# Autodesk Inventor assembly: FinalAssembly
(part 2 of 3)
590. ORingA70_.176ID_.316OD:12
## Component patterns: (4 elements, first: Bolt_ButtonHead_Hex_Thread_5_40_1inch:1), (6 elements, first: NarrowHexNutThread_5_40:5), (4 elements, first: NarrowHexNutThread_5_40:3), (6 elements, first: NarrowHexNutThread_5_40:14), (4 elements, first: ORingA50_.25OD_.125ID:24), (4 elements, first: Bolt_Buttonhead_Hex_Thread_5_40_.625inch:1), (4 elements, first: NarrowHexNutThread_5_40:20), (6 elements, first: ScrewPlastic_4_20_.75inch_Flat:1), (6 elements, first: NarrowHexNutThread_5_40:24), (2 elements), (2 elements), (2 elements), (6 elements, first: ORingA50_.25OD_.125ID:34), (6 elements, first: NarrowHexNutThread_5_40:50), (6 elements, first: aftThreadedRodThread_5_40:1), (6 elements, first: NarrowHexNutThread_5_40:56), (6 elements, first: ScrewPlastic_4_20_.75inch_Flat:19), (6 elements, first: NarrowHexNutThread_5_40:66), (3 elements, first: ScrewPlastic_4_20_.5inch:18), (6 elements, first: ORingA50_.25OD_.125ID:40), (6 elements, first: Bolt_Buttonhead_Hex_Thread_5_40_.625inch:5), (6 elements, first: NarrowHexNutThread_5_40:72), (6 elements, first: ORingA50_.25OD_.125ID:46), (2 elements), (6 elements, first: NarrowHexNutThread_5_40:84), (6 elements, first: midshipsThreadedRodThread_5_40:1), (6 elements, first: NarrowHexNutThread_5_40:90), (4 elements, first: flatPlasticScrewSmall:21), (6 elements, first: retentionStandoffs:1), (6 elements, first: NarrowHexNutThread_5_40:99), (3 elements, first: flatPlasticScrewSmall:36), (6 elements, first: ORingA50_.25OD_.125ID:52), (6 elements, first: NarrowHexNutThread_5_40:105), (6 elements, first: NarrowHexNutThread_5_40:111), (4 elements, first: ScrewPlastic_4_20_.5inch:25), (6 elements, first: NarrowHexNutThread_5_40:117), (6 elements, first: Bolt_Buttonhead_Hex_Thread_5_40_.625inch:11), (6 elements, first: flatPlasticScrewSmall:54), (3 elements, first: NarrowHexNutThread_5_40:135), (3 elements, first: NarrowHexNutThread_5_40:159), (3 elements, first: NarrowHexNutThread_5_40:165), (6 elements, first: aftServoSectionThreadedRodThread_5_40:1 + NarrowHexNutThread_5_40:175 + ORingA50_.25OD_.125ID:72 + NarrowHexNutThread_5_40:176), (6 elements, first: NarrowHexNutCaps:1), (4 elements, first: ScrewPlastic_4_20_.5inch:34), (3 elements, first: HexNutThread_M3:1), (6 elements, first: ORingA50_.25OD_.125ID:79 + Bolt_ButtonHead_Hex_Thread_5_40_1inch:5 + ORingA50_.25OD_.125ID:80), (3 elements, first: Bolt_ButtonHead_Hex_Thread_M3_10mm:1), (4 elements, first: EncoderMagnet:3), (2 elements, first: RelayModule:1), (3 elements, first: batteryHolderBracket:2), (3 elements, first: NarrowHexNutThread_5_40:216 + NarrowHexNutThread_5_40:215 + NarrowHexNutThread_5_40:218 + NarrowHexNutThread_5_40:217), (6 elements, first: NarrowHexNutThread_5_40:227), (3 elements, first: NarrowHexNutThread_5_40:233), (2 elements, first: NarrowHexNutThread_5_40:236 + NarrowHexNutThread_5_40:239 + NarrowHexNutThread_5_40:237 + NarrowHexNutThread_5_40:238), (4 elements, first: ScrewPlastic_4_20_.5inch:2), Component Pattern 27:2 (4 elements), (3 elements, first: ORingA70_.176ID_.316OD:1), Component Pattern 30:2 (3 elements), (3 elements, first: aluminumWiringTubing:1), Component Pattern 32:2 (3 elements), (3 elements, first: ORingA70_.176ID_.316OD:7), Component Pattern 50:2 (3 elements)
## Relationships (810: Mate 614, Flush 81, Angle 73, WeldJoint 21, RelateRotation 10, Tangent 6, BallJoint 4, RelateRotateTranslate 1)
- Mate:1: AftSectionAirtightRear:1 ↔ AftSectionWithSteeringLinkages:1
- Mate:5: AftSectionAirtightRear:1 ↔ aftSectionAirtightCap:2
- Mate:6: AftSectionAirtightRear:1 ↔ aftSectionAirtightCap:2
- Mate:8: AluminumSealingDisc:1 ↔ aftSectionAirtightCap:2
- Mate:10: AluminumSealingDisc:1 ↔ aftSectionAirtightCap:2
- Mate:11: AluminumSealingDisc:1 ↔ rearServoAttachmentPlate:1
- Mate:12: AluminumSealingDisc:1 ↔ rearServoAttachmentPlate:1
- Mate:13: AluminumSealingDisc:1 ↔ rearServoAttachmentPlate:1
- Mate:14: rearServoAttachmentPlate:1 ↔ HitecServoAssembly:1
- Mate:16: rearServoAttachmentPlate:1 ↔ HitecServoAssembly:1
- Mate:17: rearServoAttachmentPlate:1 ↔ HitecServoAssembly:2
- Mate:18: rearServoAttachmentPlate:1 ↔ HitecServoAssembly:2
- Mate:19: rearServoAttachmentPlate:1 ↔ HitecServoAssembly:2
- Mate:20: HitecServoAssembly:1 ↔ ServoHorn10mmPitch:1
- Mate:21: HitecServoAssembly:2 ↔ ServoHorn10mmPitch:2
- Mate:22: HitecServoAssembly:2 ↔ ServoHorn10mmPitch:2
- Mate:23: HitecServoAssembly:1 ↔ ServoHorn10mmPitch:1
- [Mate]: RearmostAftSection:2 ↔ steeringYoke3mmShaft:4
- [Mate]: RearmostAftSection:2 ↔ steeringYoke3mmShaft:3
- Mate:28 (7.747 mm): RearmostAftSection:2 ↔ steeringYoke3mmShaft:4
- Mate:29 (2.8575 mm): RearmostAftSection:2 ↔ steeringYoke3mmShaft:3
- Mate:30: AftSectionWithSteeringLinkages:1 ↔ RearmostAftSection:2
- Mate:31: AftSectionWithSteeringLinkages:1 ↔ RearmostAftSection:2
- Mate:36: ServoHorn10mmPitch:2 ↔ metalClevisis:5
- Mate:37: ServoHorn10mmPitch:1 ↔ metalClevisis:6
- Mate:55: metalClevisis:6 ↔ 2mmToServo:7
- Mate:56: metalClevisis:6 ↔ 2mmToServo:7
- Mate:59: steeringYoke3mmShaft:3 ↔ metalClevisis:7
- Mate:60 (0.762 mm): steeringYoke3mmShaft:3 ↔ metalClevisis:7
- Mate:61: steeringYoke3mmShaft:4 ↔ metalClevisis:8
- Ball:1: 2mmToDive:1 ↔ 2mmBentFromSealDive:2
- Mate:69: metalClevisis:7 ↔ 2mmBentFromSealDive:2
- Mate:70: metalClevisis:7 ↔ 2mmBentFromSealDive:2
- Ball:2: 2mmToSeal:4 ↔ 2mmToServo:8
- Mate:71: metalClevisis:5 ↔ 2mmToServo:8
- Mate:72: metalClevisis:5 ↔ 2mmToServo:8
- Ball:3: 2mmToServo:7 ↔ 2mmToSeal:5
- Ball:4: 2mmToRudder:1 ↔ 2mmBentFromSealRudder:2
- Mate:75: metalClevisis:8 ↔ 2mmBentFromSealRudder:2
- Mate:76: metalClevisis:8 ↔ 2mmBentFromSealRudder:2
- Mate:77 (0.762 mm): steeringYoke3mmShaft:4 ↔ metalClevisis:8
- Mate:101: AftSectionAirtightRear:1 ↔ aftSectionAirtightCap:2
- Mate:102: AluminumSealingDisc:1 ↔ aftSectionAirtightCap:2
- Angle:4 (10 deg): HitecServoAssembly:2 ↔ ServoHorn10mmPitch:2
- Angle:5 (-11 deg): HitecServoAssembly:1 ↔ ServoHorn10mmPitch:1
- Flush:6 (-1.016 mm): metalClevisis:8 ↔ YokeDowelPins:1
- Flush:7 (-1.016 mm): metalClevisis:7 ↔ YokeDowelPins:2
- Mate:109: RearmostAftSection:2 ↔ RudderStabilizingLowerFins:1
- Mate:110 (0.4445 mm): RearmostAftSection:2 ↔ RudderStabilizingLowerFins:1
- Mate:111: RearmostAftSection:2 ↔ RudderStabilizingLowerFins:1
- Mate:112: RearmostAftSection:2 ↔ RudderStabilizingLowerFins:2
- Mate:113: RearmostAftSection:2 ↔ RudderStabilizingLowerFins:2
- Mate:114 (0.4445 mm): RearmostAftSection:2 ↔ RudderStabilizingLowerFins:2
- Mate:118: RearmostAftSection:2 ↔ RudderStabilizingLowerFins:4
- Mate:119: RearmostAftSection:2 ↔ RudderStabilizingLowerFins:4
- Mate:120 (0.4445 mm): RearmostAftSection:2 ↔ RudderStabilizingLowerFins:4
- Mate:121: RearmostAftSection:2 ↔ SleeveBearing3mmFlanged:1
- Mate:122: RearmostAftSection:2 ↔ SleeveBearing3mmFlanged:1
- Mate:123: RearmostAftSection:2 ↔ SleeveBearing3mmFlanged:4
- Mate:124: RearmostAftSection:2 ↔ SleeveBearing3mmFlanged:4
- Mate:125: RearmostAftSection:2 ↔ SleeveBearing3mmFlanged:3
- Mate:126: RearmostAftSection:2 ↔ SleeveBearing3mmFlanged:3
- Mate:127: RearmostAftSection:2 ↔ SleeveBearing3mmFlanged:2
- Mate:128: RearmostAftSection:2 ↔ SleeveBearing3mmFlanged:2
- Mate:129: RearmostAftSection:2 ↔ DivePlanesStabilizingFins:1
- Mate:130: RearmostAftSection:2 ↔ DivePlanesStabilizingFins:2
- Mate:131: RearmostAftSection:2 ↔ DivePlanesStabilizingFins:2
- Mate:132: RearmostAftSection:2 ↔ DivePlanesStabilizingFins:2
- Mate:133: RearmostAftSection:2 ↔ DivePlanesStabilizingFins:1
- Mate:134: RearmostAftSection:2 ↔ DivePlanesStabilizingFins:1
- Mate:135: RearmostAftSection:2 ↔ RudderStabilizingFins:1
- Mate:136: RearmostAftSection:2 ↔ RudderStabilizingFins:1
- Angle:6 (0 deg): RearmostAftSection:2 ↔ RudderStabilizingFins:1
- Mate:137: RearmostAftSection:2 ↔ RudderStabilizingFinBottom:1
- Mate:138: RearmostAftSection:2 ↔ RudderStabilizingFinBottom:1
- Angle:7 (0 deg): RearmostAftSection:2 ↔ RudderStabilizingFinBottom:1
- Mate:139: SleeveBearing3mmFlanged:2 ↔ 3mmControlSurfaceShaft_1:1
- Mate:140: SleeveBearing3mmFlanged:4 ↔ 3mmControlSurfaceShaft_1:2
- Mate:141: SleeveBearing3mmFlanged:1 ↔ 3mmControlSurfaceShaft_2:1
- Mate:142: SleeveBearing3mmFlanged:3 ↔ 3mmControlSurfaceShaft_2:2
- Mate:143: 3mmControlSurfaceShaft_1:1 ↔ DivePlanesControlSurface:1
- Mate:144: 3mmControlSurfaceShaft_1:1 ↔ DivePlanesControlSurface:1
- Mate:147: 3mmControlSurfaceShaft_1:2 ↔ DivePlanesControlSurface:2
- Mate:148 (0.635 mm): DivePlanesStabilizingFins:2 ↔ DivePlanesControlSurface:2
- Mate:149: DivePlanesControlSurface:1 ↔ DivePlanesControlSurface:2
- Mate:150: 3mmControlSurfaceShaft_1:2 ↔ DivePlanesControlSurface:2
- Flush:8 (-0.762 mm): steeringYoke3mmShaft:3 ↔ 3mmControlSurfaceShaft_1:2
- Flush:9 (-0.762 mm): steeringYoke3mmShaft:3 ↔ 3mmControlSurfaceShaft_1:1
- Rigid:1 [WeldJoint] (-0.762 mm): steeringYoke3mmShaft:3 ↔ 3mmControlSurfaceShaft_1:1
- Mate:153: 3mmControlSurfaceShaft_2:1 ↔ RudderUpperControlSurface:1
- Mate:154: 3mmControlSurfaceShaft_2:1 ↔ RudderUpperControlSurface:1
- Mate:155: 3mmControlSurfaceShaft_2:2 ↔ RudderLowerControlSurface:1
- Mate:156: 3mmControlSurfaceShaft_2:2 ↔ RudderLowerControlSurface:1
- Mate:158 (0.254 mm): RudderStabilizingLowerFins:2 ↔ RudderLowerControlSurface:1
- Mate:159: RudderLowerControlSurface:1 ↔ RudderUpperControlSurface:1
- Rigid:2 [WeldJoint] (-1.016 mm): steeringYoke3mmShaft:4 ↔ 3mmControlSurfaceShaft_2:1
- Mate:160: RearmostAftSection:2 ↔ ScrewPlastic_4_20_.625inch:1
- Mate:161: RearmostAftSection:2 ↔ ScrewPlastic_4_20_.625inch:1
- Mate:162: RearmostAftSection:2 ↔ ScrewPlastic_4_20_.625inch:2
- Mate:163: RearmostAftSection:2 ↔ ScrewPlastic_4_20_.625inch:2
- Mate:164: RearmostAftSection:2 ↔ ScrewPlastic_4_20_.625inch:7
- Mate:165: RearmostAftSection:2 ↔ ScrewPlastic_4_20_.625inch:7
- Mate:166: RearmostAftSection:2 ↔ ScrewPlastic_4_20_.625inch:3
- Mate:167: RearmostAftSection:2 ↔ ScrewPlastic_4_20_.625inch:3
- Mate:168: RearmostAftSection:2 ↔ ScrewPlastic_4_20_.625inch:8
- Mate:169: RearmostAftSection:2 ↔ ScrewPlastic_4_20_.625inch:8
- Mate:170: RearmostAftSection:2 ↔ ScrewPlastic_4_20_.625inch:6
- Mate:171: RearmostAftSection:2 ↔ ScrewPlastic_4_20_.625inch:6
- Mate:190: AftSectionWithSteeringLinkages:1 ↔ NarrowHexNutThread_5_40:3
- Angle:11 (0 deg): AftSectionWithSteeringLinkages:1 ↔ NarrowHexNutThread_5_40:3
- Mate:205: AftSectionAirtightRear:1 ↔ NarrowHexNutThread_5_40:5
- Angle:13 (0 deg): AftSectionAirtightRear:1 ↔ NarrowHexNutThread_5_40:5
- Mate:206: RearmostAftSection:2 ↔ Bolt_ButtonHead_Hex_Thread_5_40_1inch:1
- Mate:216: RearmostAftSection:2 ↔ Bolt_ButtonHead_Hex_Thread_5_40_1inch:1
- Mate:219: aftSectionAirtightCap:2 ↔ NarrowHexNutThread_5_40:14
- Mate:220: aftSectionAirtightCap:2 ↔ NarrowHexNutThread_5_40:14
- Angle:14 (0 deg): aftSectionAirtightCap:2 ↔ NarrowHexNutThread_5_40:14
- Mate:221: AftSectionAirtightRear:1 ↔ MotorAssembly0:1
- Mate:223: AftSectionAirtightRear:1 ↔ MotorAssembly0:1
- Mate:224: AftSectionAirtightRear:1 ↔ Engel3mmAssembly:2
- Mate:225: AftSectionAirtightRear:1 ↔ Engel3mmAssembly:2
- Angle:15 (0 deg): AftSectionAirtightRear:1 ↔ Engel3mmAssembly:2
- Mate:226: AftSectionAirtightRear:1 ↔ Engel3mmAssembly:1
- Mate:227: AftSectionAirtightRear:1 ↔ Engel3mmAssembly:1
- Angle:16 (0 deg): AftSectionAirtightRear:1 ↔ Engel3mmAssembly:1
- Rigid:11 [WeldJoint] (-0.7937 mm): AftSectionAirtightRear:1 ↔ ORingA50_.25OD_.125ID:24
- Mate:228: AftSectionAirtightRear:1 ↔ Bolt_Buttonhead_Hex_Thread_5_40_.625inch:1
- Mate:229 (1.5875 mm): AftSectionAirtightRear:1 ↔ Bolt_Buttonhead_Hex_Thread_5_40_.625inch:1
- Mate:230: Bolt_Buttonhead_Hex_Thread_5_40_.625inch:1 ↔ NarrowHexNutThread_5_40:20
- Mate:231: MotorAssembly0:1 ↔ NarrowHexNutThread_5_40:20
- Angle:17 (0 deg): Engel3mmAssembly:1 ↔ NarrowHexNutThread_5_40:20
- Rigid:12 [WeldJoint]: AftSectionAirtightRear:1 ↔ ORingA50_1.296ID_1.574OD:1
- Tangent:1 (5.08 mm): MotorAssembly0:1 ↔ QuicrunESCAssembly:1
- Angle:18 (0 deg): HitecServoAssembly:2 ↔ QuicrunESCAssembly:1
- Flush:16 (-3.175 mm): AftSectionAirtightRear:1 ↔ QuicrunESCAssembly:1
- Flush:17 (3.048 mm): HitecServoAssembly:1 ↔ QuicrunESCAssembly:1
- Mate:244: aftSectionAirtightCap:2 ↔ ScrewPlastic_4_20_.75inch_Flat:1
- Flush:18: aftSectionAirtightCap:2 ↔ ScrewPlastic_4_20_.75inch_Flat:1
- Mate:249: rearServoAttachmentPlate:1 ↔ NarrowHexNutThread_5_40:24
- Mate:259: MotorAssembly0:1 ↔ Bolt_FlatHead_Hex_Thread_M3_8mm:2
- Mate:260: MotorAssembly0:1 ↔ Bolt_FlatHead_Hex_Thread_M3_8mm:1
- Flush:20: MotorAssembly0:1 ↔ Bolt_FlatHead_Hex_Thread_M3_8mm:1
- Flush:21: MotorAssembly0:1 ↔ Bolt_FlatHead_Hex_Thread_M3_8mm:2
- Rigid:13 [WeldJoint] (1.5875 mm): AluminumSealingDisc:1 ↔ ORingA50_3.75OD_3.5ID_Compressed:1
- Mate:261: rearServoAttachmentPlate:1 ↔ frontServoAttachmentPlate:1
- Mate:269: frontServoAttachmentPlate:1 ↔ AluminumSealingDiscMidshipsRear:1
- Mate:270: frontServoAttachmentPlate:1 ↔ AluminumSealingDiscMidshipsRear:1
- Mate:271: frontServoAttachmentPlate:1 ↔ AluminumSealingDiscMidshipsRear:1
- Mate:272: AluminumSealingDiscMidshipsRear:1 ↔ aftSpoolSectionSealingWall:1
- Mate:273: AluminumSealingDiscMidshipsRear:1 ↔ aftSpoolSectionSealingWall:1
- Mate:274: frontServoAttachmentPlate:1 ↔ aftSpoolSectionSealingWall:1
- Mate:275: rearServoAttachmentPlate:1 ↔ NarrowHexNutThread_5_40:24
- Mate:293: HitecServoAssembly:1 ↔ frontServoAttachmentPlate:1
- Mate:296: HitecServoAssembly:1 ↔ ScrewPlastic_4_20_.5inch:2
- Mate:297: HitecServoAssembly:1 ↔ ScrewPlastic_4_20_.5inch:2
- Rigid:17 [WeldJoint]: AluminumSealingDiscMidshipsRear:1 ↔ ORingA70_.176ID_.316OD:1
- Mate:300: aftSpoolSectionSealingWall:1 ↔ aluminumWiringTubing:1
- Mate:301: frontServoAttachmentPlate:1 ↔ NarrowHexNutThread_5_40:50
- Mate:302: frontServoAttachmentPlate:1 ↔ NarrowHexNutThread_5_40:50
- Mate:303: NarrowHexNutThread_5_40:50 ↔ aftThreadedRodThread_5_40:1
- Flush:25: NarrowHexNutThread_5_40:50 ↔ aftThreadedRodThread_5_40:1
- Mate:304: aftThreadedRodThread_5_40:1 ↔ NarrowHexNutThread_5_40:56
- Mate:305: aftSpoolSectionSealingWall:1 ↔ NarrowHexNutThread_5_40:56
- Mate:307: Bolt_ButtonHead_Hex_Thread_5_40_1inch:2 ↔ NarrowHexNutThread_5_40:3
- Mate:313: RearmostAftSection:2 ↔ BallBearing4mmFlanged:1
- Mate:314: RearmostAftSection:2 ↔ BallBearing4mmFlanged:1
- Mate:335: aftSpoolSectionSealingWall:1 ↔ SpoolAxle:1
- Mate:336: aftSpoolSectionSealingWall:1 ↔ SpoolAxle:1
- Mate:373: aftSpoolSectionSealingWall:1 ↔ SpoolSectionSealingWallFront:1
- Mate:374: SpoolSectionSealingWallFront:1 ↔ aftThreadedRodThread_5_40:2
- Mate:377: SpoolAxle:1 ↔ FixedCylinderWireStorage:1
- Mate:379: SpoolSectionSealingWallFront:1 ↔ FixedCylinderWireStorage:1
- Mate:380: SpoolSectionSealingWallFront:1 ↔ FixedCylinderWireStorage:1
- Mate:383: SpoolAxle:1 ↔ FixedCylinderWireStorageInsert:1
- Mate:384: FixedCylinderWireStorage:1 ↔ FixedCylinderWireStorageInsert:1
- Angle:24 (0 deg): FixedCylinderWireStorage:1 ↔ FixedCylinderWireStorageInsert:1
- Mate:385: SpoolSectionSealingWallFront:1 ↔ ScrewPlastic_4_20_.75inch_Flat:19
- Flush:52: SpoolSectionSealingWallFront:1 ↔ ScrewPlastic_4_20_.75inch_Flat:19
- Mate:386: aftThreadedRodThread_5_40:6 ↔ NarrowHexNutThread_5_40:66
- Mate:387: SpoolSectionSealingWallFront:1 ↔ NarrowHexNutThread_5_40:66
- Mate:388: SpoolSectionSealingWallFront:1 ↔ pistonTank:1
- Mate:390: SpoolSectionSealingWallFront:1 ↔ pistonTank:1
- Mate:396: pistonTank:1 ↔ pistonSealingWallFront:1
- Mate:397: pistonTank:1 ↔ pistonSealingDisc:1
- Mate:399: pistonTank:1 ↔ pistonSealingWallRear:1
- Mate:401: pistonSealingDisc:1 ↔ pistonSealingWallRear:1
- Mate:402: pistonSealingWallFront:1 ↔ pistonSealingDisc:1
- Mate:405: pistonSealingWallRear:1 ↔ ThreadedRodThread_5_16_18:1
- Mate:406: WeldNutThread_5_16_18:1 ↔ ThreadedRodThread_5_16_18:1
- Mate:407: pistonSealingWallRear:1 ↔ WeldNutThread_5_16_18:1
- Mate:408: ThreadedRodThread_5_16_18:1 ↔ HexNutThread_5_16_18:1
- Mate:409: ThreadedRodThread_5_16_18:1 ↔ WasherForThread_5_16_18:1
- Mate:410: pistonSealingWallFront:1 ↔ WasherForThread_5_16_18:1
- Mate:411: HexNutThread_5_16_18:1 ↔ WasherForThread_5_16_18:1
- Flush:53: ThreadedRodThread_5_16_18:1 ↔ HexNutThread_5_16_18:1
- Mate:412: WeldNutThread_5_16_18:1 ↔ ScrewPlastic_4_20_.5inch:18
- Mate:413: WeldNutThread_5_16_18:1 ↔ ScrewPlastic_4_20_.5inch:18
- Angle:26 (0 deg): HitecServoAssembly:1 ↔ WeldNutThread_5_16_18:1
- Rigid:20 [WeldJoint] (0.7937 mm): pistonSealingWallFront:1 ↔ ORingA50_.25OD_.125ID:40
- Mate:414: pistonSealingWallFront:1 ↔ Bolt_Buttonhead_Hex_Thread_5_40_.625inch:5
- Mate:415 (1.5875 mm): pistonSealingWallFront:1 ↔ Bolt_Buttonhead_Hex_Thread_5_40_.625inch:5
- Mate:416: Bolt_Buttonhead_Hex_Thread_5_40_.625inch:5 ↔ NarrowHexNutThread_5_40:72
- Mate:417: pistonSealingWallRear:1 ↔ NarrowHexNutThread_5_40:72
- Mate:418: pistonTank:1 ↔ forwardBallastSealingWallRear:1
- Mate:419: pistonTank:1 ↔ forwardBallastSealingWallRear:1
- Mate:420: forwardBallastSealingWallRear:1 ↔ aftThreadedRodThread_5_40:2
- Mate:421: forwardBallastSealingWallRear:1 ↔ forwardBallastSealingWallDisc:1
- Mate:422: forwardBallastSealingWallDisc:1 ↔ aftThreadedRodThread_5_40:1
- Mate:423: forwardBallastSealingWallRear:1 ↔ forwardBallastSealingWallDisc:1
- Mate:424: forwardBallastSealingWallFront:1 ↔ forwardBallastSealingWallDisc:1
- Mate:425: forwardBallastSealingWallFront:1 ↔ aftThreadedRodThread_5_40:2
- Mate:426: forwardBallastSealingWallFront:1 ↔ forwardBallastSealingWallDisc:1
- Rigid:21 [WeldJoint] (1.5875 mm): forwardBallastSealingWallDisc:1 ↔ ORingA50_3.75OD_3.5ID_Compressed:3
- Mate:427: rearServoAttachmentPlate:1 ↔ HitecServoAssembly:1
- Flush:54: AftSectionAirtightRear:1
- Flush:55: AftSectionAirtightRear:1
- Mate:428: AftSectionAirtightRear:1
- Mate:429: metalClevisis:8 ↔ YokeDowelPins:1
- Mate:430: metalClevisis:7 ↔ YokeDowelPins:2
- Mate:436: AftSectionAirtightRear:1 ↔ AftSectionWithSteeringLinkages:1
- Mate:437: AftSectionAirtightRear:1 ↔ NarrowHexNutThread_5_40:5
- Mate:438: RearmostAftSection:2 ↔ RudderStabilizingLowerFins:3
- Mate:439: RearmostAftSection:2 ↔ RudderStabilizingLowerFins:3
- Mate:440 (0.4445 mm): RearmostAftSection:2 ↔ RudderStabilizingLowerFins:3
- Mate:441: AftSectionAirtightRear:1 ↔ MotorAssembly0:1
- Rigid:23 [WeldJoint]: forwardBallastSealingWallDisc:1 ↔ ORingA70_.176ID_.316OD:7
- Mate:444: forwardBallastSealingWallFront:1 ↔ NarrowHexNutThread_5_40:84
- Mate:445: forwardBallastSealingWallFront:1 ↔ NarrowHexNutThread_5_40:84
- Angle:28 (0 deg): forwardBallastSealingWallFront:1 ↔ NarrowHexNutThread_5_40:84
- Mate:446: forwardBallastSealingWallFront:1 ↔ midshipsThreadedRodThread_5_40:1
- Mate:1021: forwardBallastSealingWallDisc:1 ↔ midshipsThreadedRodThread_5_40:1
- Mate:447: forwardBallastSealingWallFront:1 ↔ pushSwitchBushingHolder:1
- Mate:451: forwardBallastSealingWallFront:1 ↔ pushSwitchBushingHolder:1
- Mate:452: forwardBallastSealingWallFront:1 ↔ flatPlasticScrewSmall:19
- Flush:57: pushSwitchBushingHolder:1 ↔ flatPlasticScrewSmall:19
- Mate:453: forwardBallastSealingWallFront:1 ↔ flatPlasticScrewSmall:20
- Flush:58: pushSwitchBushingHolder:1 ↔ flatPlasticScrewSmall:20
- [Mate]: forwardBallastSealingWallFront:1 ↔ RadialBearingLarge:1
- [Flush]: forwardBallastSealingWallFront:1 ↔ RadialBearingLarge:1
- Mate:456: pushSwitchRod:1 ↔ pushSwitchSpring:1
- Mate:460: aftThreadedRodThread_5_40:2 ↔ NarrowHexNutThread_5_40:90
- Mate:461 (-2.54 mm): forwardBallastSealingWallFront:1 ↔ NarrowHexNutThread_5_40:90
- [Mate]: RadialBearingLarge:1 ↔ WeldNutThread_5_16_18:2
- [Flush] (1.5494 mm): RadialBearingLarge:1 ↔ WeldNutThread_5_16_18:2
- Mate:463: forwardBallastSealingWallFront:1 ↔ RadialBearingMountCover:1
- Mate:464: forwardBallastSealingWallFront:1 ↔ RadialBearingMountCover:1
- Mate:465: forwardBallastSealingWallFront:1 ↔ RadialBearingMountCover:1
- Mate:466: forwardBallastSealingWallFront:1 ↔ flatPlasticScrewSmall:21
- Flush:61 (2.032 mm): RadialBearingMountCover:1 ↔ flatPlasticScrewSmall:21
- Mate:469: RadialBearingMountCover:1 ↔ ThrustWasher:1
- Mate:470: RadialBearingMountCover:1 ↔ ThrustWasher:1
- Mate:475: midshipsThreadedRodThread_5_40:6 ↔ retentionStandoffs:1
- Mate:476: forwardBallastSealingWallFront:1 ↔ retentionStandoffs:1
- Mate:478: ThreadedRodThread_5_16_18:1 ↔ SpurGearThrustDistributer:1
- Mate:480: ThrustBearingMount:1 ↔ retentionStandoffs:2
- Mate:481: forwardBallastSealingWallFront:1 ↔ ThrustBearingMount:1
- Mate:482: ThrustBearingMount:1 ↔ retentionStandoffs:3
- Mate:485: midshipsThreadedRodThread_5_40:2 ↔ NarrowHexNutThread_5_40:99
- Mate:486: ThrustBearingMount:1 ↔ NarrowHexNutThread_5_40:99
- Mate:488: ThrustBearingMount:1 ↔ SleeveBearing.125inch:7
- Flush:490: ThrustBearingMount:1 ↔ SleeveBearing.125inch:7
- Angle:32 (0 deg): retentionStandoffs:1
- Mate:499: ThrustBearingMount:1 ↔ limitSwitchPushHolder1:1
- Mate:500: ThrustBearingMount:1 ↔ limitSwitchPushHolder1:1
- Mate:501: ThrustBearingMount:1 ↔ limitSwitchPushHolder1:1
- Mate:502: limitSwitchPushHolder1:1 ↔ flatPlasticScrewSmall:27
- Mate:503: limitSwitchPushHolder1:1 ↔ flatPlasticScrewSmall:28
- Mate:504: limitSwitchPushHolder1:1 ↔ flatPlasticScrewSmall:29
- Flush:64: limitSwitchPushHolder1:1 ↔ flatPlasticScrewSmall:27
- Flush:65: limitSwitchPushHolder1:1 ↔ flatPlasticScrewSmall:29
- Flush:66: limitSwitchPushHolder1:1 ↔ flatPlasticScrewSmall:28
- Mate:505: ThreadedRodThread_5_16_18:1 ↔ WeldNutThread_5_16_18_Cut:1
- Flush:67: ThreadedRodThread_5_16_18:1 ↔ WeldNutThread_5_16_18_Cut:1
- Angle:34 (0 deg): WeldNutThread_5_16_18_Cut:1
- Mate:506: limitSwitchPushHolder1:1 ↔ limitSwitchHolder2Backplate:1
- Mate:507: limitSwitchPushHolder1:1 ↔ limitSwitchHolder2Backplate:1
- Angle:35 (0 deg): limitSwitchPushHolder1:1 ↔ limitSwitchHolder2Backplate:1
- Mate:508: limitSwitchPushHolder1:1 ↔ flatPlasticScrewSmall:30
- Flush:68: limitSwitchHolder2Backplate:1 ↔ flatPlasticScrewSmall:30
- Mate:509: limitSwitchPushHolder1:1 ↔ LIMIT SWITCH:1
- Mate:510: limitSwitchPushHolder1:1 ↔ LIMIT SWITCH:1
- Mate:511: limitSwitchPushHolder1:1 ↔ LIMIT SWITCH:1
- Mate:512: limitSwitchPushHolder1:1 ↔ flatPlasticScrewSmall:31
- Flush:69: limitSwitchHolder2Backplate:1 ↔ flatPlasticScrewSmall:31
- Mate:513: ThrustBearingMount:1 ↔ limitSwitchHolderMount:1
- Mate:514: ThrustBearingMount:1 ↔ limitSwitchHolderMount:1
- Mate:515: ThrustBearingMount:1 ↔ limitSwitchHolderMount:1
- Mate:516: ThrustBearingMount:1 ↔ flatPlasticScrewSmall:32
- Flush:70: limitSwitchHolderMount:1 ↔ flatPlasticScrewSmall:32
- Mate:517: ThrustBearingMount:1 ↔ flatPlasticScrewSmall:33
- Flush:71: limitSwitchHolderMount:1 ↔ flatPlasticScrewSmall:33
- Mate:518: limitSwitchHolderMount:1 ↔ limitSwitchHolder2:1
- Mate:519: limitSwitchHolderMount:1 ↔ limitSwitchHolder2:1
- Mate:520: limitSwitchHolderMount:1 ↔ limitSwitchHolder2:1
- Mate:521: limitSwitchHolderMount:1 ↔ flatPlasticScrewSmall:34
- Flush:72: limitSwitchHolder2:1 ↔ flatPlasticScrewSmall:34
- Mate:522: limitSwitchHolderMount:1 ↔ flatPlasticScrewSmall:35
- Flush:73: limitSwitchHolder2:1 ↔ flatPlasticScrewSmall:35
- Mate:523: limitSwitchHolder2:1 ↔ LimitSwitchAssembly:1
- Mate:524: limitSwitchHolder2:1 ↔ LimitSwitchAssembly:1
- Mate:525: limitSwitchHolder2:1 ↔ LimitSwitchAssembly:1
- Mate:526: FixedCylinderWireStorageInsert:1 ↔ flatPlasticScrewSmall:36
- Flush:74 (0.508 mm): FixedCylinderWireStorage:1 ↔ flatPlasticScrewSmall:36
- Angle:36 (0 deg): midshipsThreadedRodThread_5_40:1
- Mate:585: forwardBallastSealingWallFront:1 ↔ foreElectronicsSealingWallRear:1
- Mate:586: foreElectronicsSealingWallRear:1 ↔ midshipsThreadedRodThread_5_40:2
- Mate:587: foreElectronicsSealingWallRear:1 ↔ foreElectronicsSealingDisc:1
- Mate:588: foreElectronicsSealingWallRear:1 ↔ foreElectronicsSealingDisc:1
- Mate:589: foreElectronicsSealingDisc:1 ↔ midshipsThreadedRodThread_5_40:2
- Mate:590: foreElectronicsSealingDisc:1 ↔ foreElectronicsSealingWallFront:1
- Mate:591: foreElectronicsSealingWallRear:1 ↔ foreElectronicsSealingWallFront:1
- Mate:592: foreElectronicsSealingWallFront:1 ↔ midshipsThreadedRodThread_5_40:2
- Flush:91 (3.175 mm): foreElectronicsSealingWallFront:1 ↔ midshipsThreadedRodThread_5_40:2
- Rigid:24 [WeldJoint] (0.7937 mm): foreElectronicsSealingWallFront:1 ↔ ORingA50_.25OD_.125ID:52
- Mate:593: midshipsThreadedRodThread_5_40:2 ↔ NarrowHexNutThread_5_40:105
- Mate:594 (0.254 mm): foreElectronicsSealingWallFront:1 ↔ NarrowHexNutThread_5_40:105
- Mate:595: midshipsThreadedRodThread_5_40:2 ↔ NarrowHexNutThread_5_40:111
- Mate:596: foreElectronicsSealingWallRear:1 ↔ NarrowHexNutThread_5_40:111
- Rigid:25 [WeldJoint] (1.524 mm): foreElectronicsSealingDisc:1 ↔ ORingA50_3.75OD_3.5ID_Compressed:4
- Angle:37 (0 deg): pistonTank:1
- Mate:597: foreElectronicsSealingWallRear:1 ↔ HitecServoAssembly:3
- Mate:598: foreElectronicsSealingWallRear:1 ↔ HitecServoAssembly:3
- Angle:38 (0 deg): foreElectronicsSealingWallRear:1 ↔ HitecServoAssembly:3
- Mate:599: HitecServoAssembly:3 ↔ ScrewPlastic_4_20_.5inch:25
- Mate:600: HitecServoAssembly:3 ↔ ScrewPlastic_4_20_.5inch:25
- Mate:601: foreElectronicsSealingWallFront:1 ↔ foreElectronicsSealingWallFrontCap:1
- Flush:92: foreElectronicsSealingWallFront:1 ↔ foreElectronicsSealingWallFrontCap:1
- Flush:93: foreElectronicsSealingWallFront:1 ↔ foreElectronicsSealingWallFrontCap:1
- Mate:611: foreElectronicsSealingWallFront:1 ↔ SleeveBearing3mm:4
- Mate:612: foreElectronicsSealingWallFront:1 ↔ SleeveBearing3mm:4
- Mate:613: foreElectronicsSealingWallFront:1 ↔ SleeveBearing3mm:5
- Mate:614: foreElectronicsSealingWallFront:1 ↔ SleeveBearing3mm:5
- Mate:615: foreElectronicsSealingWallFront:1 ↔ Engel3mmAssembly:5
- Mate:616: foreElectronicsSealingWallFront:1 ↔ Engel3mmAssembly:5
- Angle:39 (0 deg): foreElectronicsSealingWallFront:1 ↔ Engel3mmAssembly:5
- Mate:617: foreElectronicsSealingWallFront:1 ↔ Engel3mmAssembly:6
- Mate:618: foreElectronicsSealingWallFront:1 ↔ Engel3mmAssembly:6
- Angle:40 (0 deg): foreElectronicsSealingWallFront:1 ↔ Engel3mmAssembly:6
- Mate:619: 3mmControlSurfaceShaftForePlanes:1 ↔ foreDivePlanes:1
- Mate:620: 3mmControlSurfaceShaftForePlanes:1 ↔ foreDivePlanes:1
- Mate:621: 3mmControlSurfaceShaftForePlanes:2 ↔ foreDivePlanes:2
- Mate:622: 3mmControlSurfaceShaftForePlanes:2 ↔ foreDivePlanes:2
- Mate:623: SleeveBearing3mm:4 ↔ 3mmControlSurfaceShaftForePlanes:1
- Mate:624: SleeveBearing3mm:5 ↔ 3mmControlSurfaceShaftForePlanes:2
- Tangent:2 (3.175 mm): foreElectronicsSealingWallFront:1 ↔ foreDivePlanes:2
- Tangent:3 (3.175 mm): foreElectronicsSealingWallFront:1 ↔ foreDivePlanes:1
- Flush:103: foreDivePlanes:1 ↔ foreDivePlanes:2
- Mate:625: 3mmControlSurfaceShaftForePlanes:2 ↔ steeringYoke3mmShaft:5
- Mate:626 (1.905 mm): foreElectronicsSealingWallFront:1 ↔ steeringYoke3mmShaft:5
- Angle:41 (88 deg): foreDivePlanes:2 ↔ steeringYoke3mmShaft:5
- Mate:627: HitecServoAssembly:3 ↔ ServoHorn10mmPitch:3
- Mate:628: HitecServoAssembly:3 ↔ ServoHorn10mmPitch:3
- Mate:629: ServoHorn10mmPitch:3 ↔ foreDivePlanesLinkage:2
- Mate:630: steeringYoke3mmShaft:5 ↔ foreDivePlanesLinkage:2
- Tangent:4 (0.762 mm): ServoHorn10mmPitch:3 ↔ foreDivePlanesLinkage:2
- Mate:631: foreElectronicsSealingWallFront:1 ↔ NarrowHexNutThread_5_40:117
- Mate:632: foreElectronicsSealingWallFront:1 ↔ NarrowHexNutThread_5_40:117
- Angle:42 (0 deg): foreElectronicsSealingWallFront:1 ↔ NarrowHexNutThread_5_40:117
- Mate:633: foreElectronicsSealingWallFront:1 ↔ foreHullLower:1
- Mate:634: foreElectronicsSealingWallFront:1 ↔ foreHullLower:1
- Mate:635: foreElectronicsSealingWallFront:1 ↔ foreHullLower:1
- Mate:636: foreHullLower:1 ↔ Bolt_Buttonhead_Hex_Thread_5_40_.625inch:11
- Mate:637: foreHullLower:1 ↔ Bolt_Buttonhead_Hex_Thread_5_40_.625inch:11
- Mate:638: foreHullInsert:1 ↔ foreHullUpper:1
- Mate:639: foreHullInsert:1 ↔ foreHullUpper:1
- Mate:640: foreHullInsert:1 ↔ foreHullUpper:1
- Mate:641: foreHullLower:1 ↔ foreHullUpper:1
- Mate:642: foreElectronicsSealingWallFront:1 ↔ foreHullInsert:1
- Angle:43 (0 deg): foreHullUpper:1
- Mate:643: foreHullInsert:1 ↔ flatPlasticScrewSmall:54
- Flush:104: foreHullInsert:1 ↔ flatPlasticScrewSmall:54
- Mate:644: ArduinoMegaHolder1:1 ↔ midshipsThreadedRodThread_5_40:1
- Mate:645: ArduinoMegaHolder1:1 ↔ midshipsThreadedRodThread_5_40:2
- Mate:646: ArduinoMegaHolder2:1 ↔ midshipsThreadedRodThread_5_40:1
- Mate:647: ArduinoMegaHolder2:1 ↔ midshipsThreadedRodThread_5_40:3
- Mate:648: ArduinoMegaHolder1:1 ↔ ArduinoMega:1
- Mate:649: ArduinoMegaHolder2:1 ↔ ArduinoMega:1
- Mate:650: ArduinoMegaHolder1:1 ↔ ArduinoMega:1
- Mate:651 (0.889 mm): ArduinoMegaHolder2:1 ↔ ArduinoMega:1
- Mate:654: ServoControllerHolder:1 ↔ ServoControllerHolder:2
- Mate:655: ServoControllerHolder:1 ↔ midshipsThreadedRodThread_5_40:2
- Mate:656: ServoControllerHolder:1 ↔ ServoControllerHolder:2
- Mate:657: ServoControllerHolder:1 ↔ midshipsThreadedRodThread_5_40:6
- Mate:658: ServoControllerHolder:1 ↔ ServoControllerAssembly:1
- Mate:659: ServoControllerHolder:1 ↔ ServoControllerAssembly:1
- Mate:660 (0.508 mm): ServoControllerHolder:1 ↔ ServoControllerAssembly:1
- Mate:661: ServoControllerHolder:2 ↔ ServoControllerAssembly:1
- Mate:662: midshipsThreadedRodThread_5_40:2 ↔ NarrowHexNutThread_5_40:135
- Mate:663: ServoControllerHolder:1 ↔ NarrowHexNutThread_5_40:135
- Mate:664: ArduinoNanoHolderSide2:1 ↔ midshipsThreadedRodThread_5_40:6
- Mate:665: ArduinoNanoHolderSide2:1 ↔ midshipsThreadedRodThread_5_40:1
- Mate:666: ArduinoNanoHolder:1 ↔ midshipsThreadedRodThread_5_40:1
- Mate:667: ArduinoNanoHolder:1 ↔ midshipsThreadedRodThread_5_40:6
- Mate:668: ArduinoNanoHolder:1 ↔ ArduinoNanoHolderSide2:1
- Mate:672: ArduinoNanoHolderSide2:1 ↔ ArduinoNanoNoPins:1
- Flush:105: ArduinoNanoHolder:1 ↔ ArduinoNanoNoPins:1
- Flush:106: ArduinoNanoHolder:1 ↔ ArduinoNanoNoPins:1
- Mate:673: NarrowHexNutThread_5_40:147 ↔ midshipsThreadedRodThread_5_40:6
- Mate:674: ArduinoNanoHolderSide2:1 ↔ NarrowHexNutThread_5_40:147
- Mate:675: NarrowHexNutThread_5_40:148 ↔ midshipsThreadedRodThread_5_40:6
- Mate:676: ArduinoNanoHolderSide2:1 ↔ NarrowHexNutThread_5_40:148
- Mate:681: NarrowHexNutThread_5_40:151 ↔ midshipsThreadedRodThread_5_40:6
- Mate:682: ArduinoNanoHolder:1 ↔ NarrowHexNutThread_5_40:151
- Mate:685 (30.48 mm): foreElectronicsSealingWallRear:1 ↔ ArduinoMegaHolder1:1
- Mate:686: ArduinoMegaHolder2:1 ↔ ArduinoNanoHolderSide2:1
- Mate:687: ArduinoMegaHolder2:1 ↔ ServoControllerHolder:2
- Mate:688: midshipsThreadedRodThread_5_40:3 ↔ NarrowHexNutThread_5_40:159
- Mate:689: ArduinoMegaHolder1:1 ↔ NarrowHexNutThread_5_40:159
- Mate:690: midshipsThreadedRodThread_5_40:3 ↔ NarrowHexNutThread_5_40:165
- Mate:691: ArduinoMegaHolder1:1 ↔ NarrowHexNutThread_5_40:165
- Mate:692: NarrowHexNutThread_5_40:168 ↔ midshipsThreadedRodThread_5_40:3
- Mate:693: ArduinoMegaHolder2:1 ↔ NarrowHexNutThread_5_40:168
- Mate:694: NarrowHexNutThread_5_40:169 ↔ midshipsThreadedRodThread_5_40:2
- Mate:695: ArduinoMegaHolder2:1 ↔ NarrowHexNutThread_5_40:169
- Tangent:5 (1.27 mm): QuicrunESCAssembly:2 ↔ midshipsThreadedRodThread_5_40:2
- Angle:44 (0 deg): ArduinoMega:1 ↔ QuicrunESCAssembly:2
- Angle:45 (0 deg): HitecServoAssembly:3 ↔ QuicrunESCAssembly:2
- Mate:698 (7.62 mm): limitSwitchPushHolder1:1 ↔ QuicrunESCAssembly:2
- Flush:108 (-13.97 mm): HitecServoAssembly:3 ↔ QuicrunESCAssembly:2
- Tangent:6: BEC_Assembly:1 ↔ midshipsThreadedRodThread_5_40:3
- Flush:109: limitSwitchPushHolder1:1 ↔ BEC_Assembly:1
- Mate:700: AftSectionAirtightRear:1 ↔ PrimaryHullLexanTube_01:1
- Mate:701: aftSectionAirtightCap:2 ↔ PrimaryHullLexanTube_01:1
- Angle:46 (0 deg): PrimaryHullLexanTube_01:1
- Mate:702: foreHullUpper:1 ↔ 5mmLED:1
- Flush:110 (12.7 mm): foreHullInsert:1 ↔ 5mmLED:1
- Mate:703: foreHullUpper:1 ↔ 5mmLED:2
- Flush:111: 5mmLED:1 ↔ 5mmLED:2
- Mate:706: metalClevisis:6 ↔ YokeDowelPins:4
- Flush:112 (-0.762 mm): metalClevisis:6 ↔ YokeDowelPins:4
- Mate:707: metalClevisis:5 ↔ YokeDowelPins:3
- Flush:113 (-0.762 mm): metalClevisis:5 ↔ YokeDowelPins:3
- Mate:713: ServoWithShaftAssembly:1 ↔ PinionGear:1
- Mate:734 (35.56 mm): ThrustBearingMount:1 ↔ BEC_Assembly:1
- Angle:49 (185 deg): foreElectronicsSealingWallFrontCap:1 ↔ ElectronicsBatteryAssembly:1
- Flush:117 (-30.48 mm): ElectronicsBatteryAssembly:1
- Mate:736: PrimaryHullLexanTube_01:1 ↔ SailAssembly:1
- Angle:52 (0 deg): SailAssembly:1
- Mate:737 (-177.8 mm): PrimaryHullLexanTube_01:1 ↔ SailAssembly:1
- Mate:738 (45.72 mm): foreElectronicsSealingWallFront:1 ↔ PressureSensor:2
- Angle:53 (0 deg): HitecServoAssembly:3 ↔ PressureSensor:2
- Mate:739: PressureSensor:2
- Flush:118 (-13.97 mm): HitecServoAssembly:3 ↔ PressureSensor:2
- Mate:802: PrimaryHullLexanTube_01:1 ↔ WireGuide:1
- Mate:803: PrimaryHullLexanTube_01:1 ↔ WireGuide:2
- Mate:804: PrimaryHullLexanTube_01:1 ↔ WireGuideToSail1:1
- Mate:805: SailAssembly:1 ↔ WireGuideToSail1:1
- Mate:806: WireGuide:1 ↔ WireGuideToSail1:1
- Mate:807: SailAssembly:1 ↔ WireGuideToSail1:1
- Mate:808: SailAssembly:1 ↔ WireGuide:1
- Mate:812: SailAssembly:1 ↔ WireGuide:2
- Mate:813: PrimaryHullLexanTube_01:1 ↔ WireGuideToSail2:1
- Mate:814: SailAssembly:1 ↔ WireGuideToSail2:1
- Mate:815: WireGuide:2 ↔ WireGuideToSail2:1
- Mate:816: SailAssembly:1 ↔ WireGuideToSail2:1
- Mate:817: PrimaryHullLexanTube_01:1 ↔ WireGuideToMiniSub:1
- Mate:818: WireGuide:2 ↔ WireGuideToMiniSub:1
- Mate:819: WireGuideToSail2:1 ↔ WireGuideToMiniSub:1
- Mate:820: PrimaryHullLexanTube_01:1 ↔ WireGuideToMiniSubExtender:1
- Mate:821: WireGuideToMiniSub:1 ↔ WireGuideToMiniSubExtender:1
- Mate:822: WireGuideToMiniSub:1 ↔ WireGuideToMiniSubExtender:1
- Mate:826: SpoolAxle:1 ↔ SmallSpoolAssembly:1
- Mate:827 (16.51 mm): aftSpoolSectionSealingWall:1 ↔ SmallSpoolAssembly:1
- Flush:120: PinionGear:1 ↔ SmallSpoolAssembly:1
- Mate:828: aftSpoolSectionSealingWall:1 ↔ CarriageImproved:1
- Mate:829: aftSpoolSectionSealingWall:1 ↔ CarriageImproved:1
- Mate:830: frontServoAttachmentPlate:1 ↔ SleeveBearing.125inch:8
- Mate:831: frontServoAttachmentPlate:1 ↔ SleeveBearing.125inch:8
- Mate:836: frontServoAttachmentPlate:1 ↔ MiniSpoolServoShaft:1
- Mate:837: aftSpoolSectionSealingWall:1 ↔ SleeveBearing.125inch:9
- Mate:838: aftSpoolSectionSealingWall:1 ↔ SleeveBearing.125inch:9
- Rigid:28 [WeldJoint]: AluminumSealingDiscMidshipsRear:1 ↔ ORingA50_.25OD_.125ID:70
- Mate:839: frontServoAttachmentPlate:1 ↔ CarriageConnectorShaft:1
- Mate:840: frontServoAttachmentPlate:1 ↔ SleeveBearing.125inch:10
- Flush:122: frontServoAttachmentPlate:1 ↔ SleeveBearing.125inch:10
- Mate:841: MiniSpoolServoShaft:1 ↔ smallIdlerPinion:7
- Mate:843: CarriageConnectorShaft:1 ↔ largeIdlerPinion:4
- Mate:845: aftSpoolSectionSealingWall:1 ↔ carriageRideShaft:1
- Mate:846: AluminumSealingDiscMidshipsRear:1 ↔ carriageRideShaft:1
- Mate:847: aftSpoolSectionSealingWall:1 ↔ spoolCarriageThreadedRodThread_5_40:1
- Mate:848: AluminumSealingDiscMidshipsRear:1 ↔ spoolCarriageThreadedRodThread_5_40:1
- Mate:849: aftSpoolSectionSealingWall:1 ↔ bearing_1_8inch:14
- Flush:124: aftSpoolSectionSealingWall:1 ↔ bearing_1_8inch:14
- Mate:850: CarriageImproved:1 ↔ SleeveBearing.125inch:11
- Mate:851: CarriageImproved:1 ↔ SleeveBearing.125inch:11
- Mate:852: CarriageImproved:1 ↔ SleeveBearing.125inch:12
- Mate:853: CarriageImproved:1 ↔ SleeveBearing.125inch:12
- Mate:854: CarriageImproved:1 ↔ NarrowHexNutThread_5_40:174
- Mate:855: CarriageImproved:1 ↔ NarrowHexNutThread_5_40:174
- Angle:58 (0 deg): CarriageImproved:1 ↔ NarrowHexNutThread_5_40:174
- Mate:856: CarriageImproved:1 ↔ NarrowHexNutThread_5_40:173
- Mate:857: CarriageImproved:1 ↔ NarrowHexNutThread_5_40:173
- Angle:59 (0 deg): CarriageImproved:1 ↔ NarrowHexNutThread_5_40:173
- Mate:858: rearServoAttachmentPlate:1 ↔ aftServoSectionThreadedRodThread_5_40:1
- Flush:125: NarrowHexNutThread_5_40:19 ↔ aftServoSectionThreadedRodThread_5_40:1
- Mate:859: aftServoSectionThreadedRodThread_5_40:1 ↔ NarrowHexNutThread_5_40:175
- Mate:860: frontServoAttachmentPlate:1 ↔ NarrowHexNutThread_5_40:175
- Mate:861: aftServoSectionThreadedRodThread_5_40:1 ↔ NarrowHexNutThread_5_40:176
- Flush:126 (1.27 mm): aftServoSectionThreadedRodThread_5_40:1 ↔ NarrowHexNutThread_5_40:176
- Mate:864: spoolCarriageThreadedRodThread_5_40:1 ↔ PinionGear20T:1
- Mate:865 (2.54 mm): aftSpoolSectionSealingWall:1 ↔ PinionGear20T:1
- Mate:866: aftSpoolSectionSealingWall:1 ↔ SleeveBearing.125inch:13
- Flush:127: aftSpoolSectionSealingWall:1 ↔ SleeveBearing.125inch:13
- Mate:867: CarriageConnectorShaft:1 ↔ smallIdlerPinion:8
- Flush:129: PinionGear20T:1 ↔ smallIdlerPinion:8
- Mate:876: CarrageRodEndMount:1 ↔ aftThreadedRodThread_5_40:1
- Mate:877: CarrageRodEndMount:1 ↔ aftThreadedRodThread_5_40:2
- Mate:878: CarrageRodEndMount:1 ↔ bearing_1_8inch:15
- Mate:879: CarrageRodEndMount:1 ↔ bearing_1_8inch:15
- Mate:880: spoolCarriageThreadedRodThread_5_40:1 ↔ CarrageRodEndMount:1
- Mate:881: NarrowHexNutThread_5_40:187 ↔ aftThreadedRodThread_5_40:1
- Mate:882: CarrageRodEndMount:1 ↔ NarrowHexNutThread_5_40:187
- Mate:883: NarrowHexNutThread_5_40:188 ↔ aftThreadedRodThread_5_40:1
- Mate:884: CarrageRodEndMount:1 ↔ NarrowHexNutThread_5_40:188
- Mate:885: CarrageRodEndMount:1 ↔ NarrowHexNutThread_5_40:189
- Mate:886: NarrowHexNutThread_5_40:189 ↔ aftThreadedRodThread_5_40:2
- Mate:887: NarrowHexNutThread_5_40:190 ↔ aftThreadedRodThread_5_40:2
- Mate:888: CarrageRodEndMount:1 ↔ NarrowHexNutThread_5_40:190
- Rigid:31 [WeldJoint]: AluminumSealingDiscMidshipsRear:1 ↔ ORingA50_.25OD_.125ID:71
- Rigid:32 [WeldJoint] (-1.524 mm): AluminumSealingDiscMidshipsRear:1 ↔ ORingA50_3.75OD_3.5ID_Compressed:2
- Mate:889: AluminumSealingDiscMidshipsRear:1 ↔ ServoWithShaftAssembly:1
- Angle:61 (0 deg): QuicrunESCAssembly:1 ↔ ServoWithShaftAssembly:1
- Mate:890: SpoolServoMount:1 ↔ aftServoSectionThreadedRodThread_5_40:2
- Mate:891: SpoolServoMount:1 ↔ aftServoSectionThreadedRodThread_5_40:4
- Mate:892: ServoWithShaftAssembly:1 ↔ SpoolServoMount:1
- Mate:893: ServoWithShaftAssembly:1 ↔ ScrewPlastic_4_20_.5inch:32
- Mate:894: ServoWithShaftAssembly:1 ↔ ScrewPlastic_4_20_.5inch:32
- Mate:895: ServoWithShaftAssembly:1 ↔ ScrewPlastic_4_20_.5inch:33
- Mate:896: ServoWithShaftAssembly:1 ↔ ScrewPlastic_4_20_.5inch:33
- Mate:897: NarrowHexNutThread_5_40:191 ↔ aftServoSectionThreadedRodThread_5_40:4
- Mate:898: SpoolServoMount:1 ↔ NarrowHexNutThread_5_40:191
- Mate:899: NarrowHexNutThread_5_40:192 ↔ aftServoSectionThreadedRodThread_5_40:4
- Mate:900: SpoolServoMount:1 ↔ NarrowHexNutThread_5_40:192
- Mate:905: NarrowHexNutThread_5_40:196 ↔ aftServoSectionThreadedRodThread_5_40:2
- Mate:906: SpoolServoMount:1 ↔ NarrowHexNutThread_5_40:196
- Mate:907: NarrowHexNutThread_5_40:197 ↔ aftServoSectionThreadedRodThread_5_40:2
- Mate:908: SpoolServoMount:1 ↔ NarrowHexNutThread_5_40:197
- Flush:130: ServoWithShaftAssembly:1 ↔ PinionGear:1
- Rigid:33 [WeldJoint] (1.8415 mm): pistonSealingDisc:1 ↔ ORingA70_2.484ID_2.762OD_Compressed:1
- Mate:914: pistonSealingWallRear:1 ↔ SleeveBearing.125inch:15
- Flush:132: pistonSealingWallRear:1 ↔ SleeveBearing.125inch:15
- Rigid:34 [WeldJoint]: pistonSealingDisc:1 ↔ ORingA50_.25OD_.125ID:78
- Mate:915: NarrowHexNutThread_5_40:110 ↔ NarrowHexNutCaps:1
- Mate:916 (0.127 mm): NarrowHexNutThread_5_40:110 ↔ NarrowHexNutCaps:1
- Mate:917 (0.127 mm): NarrowHexNutThread_5_40:110 ↔ NarrowHexNutCaps:1
- Mate:921: MotorAssembly0:1 ↔ 4mmShaftCollar:1
- Mate:929: 4mmShaftCollar:1 ↔ ShaftCollarMagnetMount:1
- Mate:930: 4mmShaftCollar:1 ↔ ShaftCollarMagnetMount:1
- Mate:931: ShaftCollarMagnetMount:1 ↔ EncoderMagnet:2
- Flush:138: ShaftCollarMagnetMount:1 ↔ EncoderMagnet:2
- Mate:932: ShaftCollarMagnetMount:1 ↔ EncoderMagnet:1
- Flush:139: ShaftCollarMagnetMount:1 ↔ EncoderMagnet:1
- Mate:965: ThrustBearingMount:1 ↔ bearing_1_8inch:19
- Flush:146: ThrustBearingMount:1 ↔ bearing_1_8inch:19
- Mate:966: ThrustBearingMount:1 ↔ bearing_1_8inch:20
- Flush:147: ThrustBearingMount:1 ↔ bearing_1_8inch:20
- Mate:967: ThrustBearingMount:1 ↔ bearing_1_8inch:21
- Flush:148: ThrustBearingMount:1 ↔ bearing_1_8inch:21
- Mate:968: ThrustBearingMount:1 ↔ idlerShaftBearingMount:1
- Mate:969: ThrustBearingMount:1 ↔ idlerShaftBearingMount:1
- Mate:970: ThrustBearingMount:1 ↔ idlerShaftBearingMount:1
- Mate:971: 540DCMotor:1 ↔ idlerShaftBearingMount:1
- Mate:972: 540DCMotor:1 ↔ idlerShaftBearingMount:1
- Mate:973: 540DCMotor:1 ↔ idlerShaftBearingMount:1
- Mate:974: ThrustBearingMount:1 ↔ BearingRetentionBrace:1
- Mate:975: ThrustBearingMount:1 ↔ BearingRetentionBrace:1
- Mate:976: ThrustBearingMount:1 ↔ BearingRetentionBrace:1
- Mate:977: 540DCMotor:1 ↔ smallIdlerPinion:9
- Mate:978 (0.381 mm): 540DCMotor:1 ↔ smallIdlerPinion:9
- Mate:979: bearing_1_8inch:16 ↔ idlerShaft:1
- Flush:149: forwardBallastSealingWallFront:1 ↔ aftThreadedRodThread_5_40:2
- Mate:981: bearing_1_8inch:17 ↔ idlerShaft2:1
- Mate:983: bearing_1_8inch:18 ↔ idlerShaft2:2
- Mate:985: idlerShaft:1 ↔ largeIdlerPinion:5
- Flush:150: smallIdlerPinion:9 ↔ largeIdlerPinion:5
- Mate:986: idlerShaft:1 ↔ smallIdlerPinion:10
- Mate:987: idlerShaft2:1 ↔ largeIdlerPinion:6
- Mate:988: idlerShaft2:1 ↔ smallIdlerPinion:11
- Mate:989: idlerShaft2:2 ↔ largeIdlerPinion:7
- Mate:990: idlerShaft2:2 ↔ smallIdlerPinion:12
- Flush:151: largeIdlerPinion:6 ↔ smallIdlerPinion:10
- Flush:152: largeIdlerPinion:7 ↔ smallIdlerPinion:11
- Mate:992 (0.381 mm): ThrustBearingMount:1 ↔ smallIdlerPinion:11
- Mate:993 (0.635 mm): largeIdlerPinion:7 ↔ smallIdlerPinion:12
- Mate:994: NarrowHexNutThread_5_40:201 ↔ midshipsThreadedRodThread_5_40:2
- Mate:995: ServoControllerHolder:2 ↔ NarrowHexNutThread_5_40:201
- Rigid:35 [WeldJoint] (0.762 mm): frontServoAttachmentPlate:1 ↔ ORingA50_.25OD_.125ID:34
- Flush:153 (3.81 mm): forwardBallastSealingWallFront:1 ↔ aluminumWiringTubing:1
- Rigid:36 [WeldJoint] (0.762 mm): aftSpoolSectionSealingWall:1 ↔ ORingA50_.25OD_.125ID:72
- Rigid:37 [WeldJoint] (0.762 mm): forwardBallastSealingWallFront:1 ↔ ORingA50_.25OD_.125ID:46
- Mate:997: BearingRetentionBrace:1 ↔ flatPlasticScrewSmall:64
- Flush:154: BearingRetentionBrace:1 ↔ flatPlasticScrewSmall:64
- Mate:998: BearingRetentionBrace:1 ↔ flatPlasticScrewSmall:65
- Flush:155: BearingRetentionBrace:1 ↔ flatPlasticScrewSmall:65
- Mate:999: ThrustBearingMount:1 ↔ Bolt_SocketHead_Hex_Thread_M3_16mm:1
- Mate:1000: ThrustBearingMount:1 ↔ Bolt_SocketHead_Hex_Thread_M3_16mm:1
- Mate:1001: ThrustBearingMount:1 ↔ Bolt_SocketHead_Hex_Thread_M3_16mm:2
- Mate:1002: ThrustBearingMount:1 ↔ Bolt_SocketHead_Hex_Thread_M3_16mm:2
- Mate:1003: ThrustBearingMount:1 ↔ ScrewPlastic_4_20_.5inch:34
- Mate:1004: ThrustBearingMount:1 ↔ ScrewPlastic_4_20_.5inch:34
- Rotation:1 [RelateRotation] (0.5714 ul): largeIdlerPinion:7 ↔ smallIdlerPinion:11
- Rotation:2 [RelateRotation] (0.5714 ul): largeIdlerPinion:6 ↔ smallIdlerPinion:10
- Rotation:3 [RelateRotation] (0.5714 ul): smallIdlerPinion:9 ↔ largeIdlerPinion:5
- Rotation:4 [RelateRotation] (1 ul): idlerShaft:1 ↔ largeIdlerPinion:5
- Rotation:5 [RelateRotation] (1 ul): idlerShaft:1 ↔ smallIdlerPinion:10
- Rotation:6 [RelateRotation] (1 ul): idlerShaft2:1 ↔ smallIdlerPinion:11
- Rotation:7 [RelateRotation] (1 ul): idlerShaft2:1 ↔ largeIdlerPinion:6
- Rotation:8 [RelateRotation] (1 ul): idlerShaft2:2 ↔ largeIdlerPinion:7
- Rotation:9 [RelateRotation] (1 ul): idlerShaft2:2 ↔ smallIdlerPinion:12
- Mate:1005: ThreadedRodThread_5_16_18:1 ↔ pistonSpurGear:1
- Mate:1006: ThrustWasher:1 ↔ pistonSpurGear:1
- Mate:1007: ThrustWasher:1 ↔ CompressionWasherPlastic:1
- Mate:1008: WeldNutThread_5_16_18:2 ↔ CompressionWasherPlastic:1
- Angle:63 (30.1 deg): WeldNutThread_5_16_18:2 ↔ CompressionWasherPlastic:1
- Mate:1012: pistonSpurGear:1 ↔ HexNutThread_M3:1
- Angle:64 (60 deg): WeldNutThread_5_16_18:2 ↔ pistonSpurGear:1
- Mate:1013: SpurGearThrustDistributer:1 ↔ pistonSpurGear:1
- Angle:65 (0 deg): SpurGearThrustDistributer:1 ↔ pistonSpurGear:1
- Mate:1014: ThrustBearingMount:1 ↔ ThrustWasherPrimary:1
- Mate:1015: ThrustBearingMount:1 ↔ ThrustWasherPrimary:1
- Rotation:10 [RelateRotation] (0.1882 ul): smallIdlerPinion:12 ↔ pistonSpurGear:1
- Rotation/Translation:1 [RelateRotateTranslate] (2.54 mm): ThreadedRodThread_5_16_18:1 ↔ pistonSpurGear:1
- Mate:1022: pushSwitchRod:1 ↔ smallIdlerPinion:13
- Mate:1023: pushSwitchSpring:1 ↔ ThrustBearingMount:1
- Mate:1024 (15.494 mm): ThrustBearingMount:1 ↔ smallIdlerPinion:13
- Mate:1025: pushSwitchRod:1 ↔ pushSwitchRodSpacer:1
- Mate:1026: smallIdlerPinion:13 ↔ pushSwitchRodSpacer:1
- Mate:1027: ThrustBearingMount:1 ↔ ThrustWasherPrimary:2
- Mate:1028: ThrustWasherPrimary:1 ↔ ThrustWasherPrimary:2
- Mate:1029: MotorAssembly0:1 ↔ ScimitarPropellerModel1:1
- Mate:1030: BallBearing4mmFlanged:1 ↔ ScimitarPropellerModel1:1
- Mate:1031: AftSectionWithSteeringLinkages:1 ↔ Bolt_ButtonHead_Hex_Thread_5_40_1inch:5
- Flush:491: NarrowHexNutThread_5_40:5 ↔ Bolt_ButtonHead_Hex_Thread_5_40_1inch:5
- Rigid:38 [WeldJoint]: AftSectionWithSteeringLinkages:1 ↔ ORingA50_.25OD_.125ID:79
- Rigid:39 [WeldJoint]: AftSectionWithSteeringLinkages:1 ↔ ORingA50_.25OD_.125ID:80
- Mate:1033: SleeveBearing.125inch:8 ↔ MiniSpoolServoShaft:1
- Mate:1034: MiniSpoolServoShaft:1 ↔ 3mm_.125inch_ShaftCoupler:1
- Mate:1037: GearMotorMount:1 ↔ aftServoSectionThreadedRodThread_5_40:6
- Angle:66 (0 deg): aftServoSectionThreadedRodThread_5_40:1
- Mate:1039: GearMotorMount:1 ↔ MicroGearMotor:1
- Mate:1040: 3mm_.125inch_ShaftCoupler:1 ↔ MicroGearMotor:1
- Angle:67 (0 deg): GearMotorMount:1 ↔ MicroGearMotor:1
- Mate:1041 (2.54 mm): 3mm_.125inch_ShaftCoupler:1 ↔ GearMotorMount:1
- Angle:68 (0 deg): 3mm_.125inch_ShaftCoupler:1
- Mate:1042: NarrowHexNutThread_5_40:202 ↔ aftServoSectionThreadedRodThread_5_40:6
- Mate:1043: GearMotorMount:1 ↔ NarrowHexNutThread_5_40:202
- Mate:1044: NarrowHexNutThread_5_40:203 ↔ aftServoSectionThreadedRodThread_5_40:6
- Mate:1045: GearMotorMount:1 ↔ NarrowHexNutThread_5_40:203
- Angle:69 (0 deg): MicroGearMotor:1 ↔ NarrowHexNutThread_5_40:203
- Mate:1046: NarrowHexNutThread_5_40:204 ↔ aftServoSectionThreadedRodThread_5_40:1
- Mate:1047: GearMotorMount:1 ↔ NarrowHexNutThread_5_40:204
- Mate:1048: NarrowHexNutThread_5_40:205 ↔ aftServoSectionThreadedRodThread_5_40:1
- Mate:1049: NarrowHexNutThread_5_40:205 ↔ GearMotorMountArm:1
- Angle:70 (0 deg): HitecServoAssembly:2 ↔ NarrowHexNutThread_5_40:24
- Mate:1059: PrimaryHullLexanTube_01:1 ↔ ASDSAttachmentAssemblyUpdated:1
- Angle:71 (0 deg): ASDSAttachmentAssemblyUpdated:1
- Mate:1061: AftSectionWithSteeringLinkages:1 ↔ hallEffectSensorAssembly:1
- Mate:1062: AftSectionWithSteeringLinkages:1 ↔ hallEffectSensorAssembly:1
- Mate:1063: AftSectionWithSteeringLinkages:1 ↔ hallEffectSensorAssembly:1
- Mate:1064: AftSectionWithSteeringLinkages:1 ↔ flatPlasticScrewSmall:66
- Mate:1065: AftSectionWithSteeringLinkages:1 ↔ flatPlasticScrewSmall:67
- Flush:494 (-4.445 mm): hallEffectSensorAssembly:1 ↔ flatPlasticScrewSmall:66
- Flush:495 (-4.445 mm): hallEffectSensorAssembly:1 ↔ flatPlasticScrewSmall:67
- Angle:73 (0 deg): forwardBallastSealingWallFront:1 ↔ NarrowHexNutThread_5_40:90
- Mate:1072: forwardBallastSealingWallFront:1 ↔ gearboxBearingHolderForward:1
- Mate:1073: gearboxBearingHolderForward:1
- Mate:1074: forwardBallastSealingWallFront:1 ↔ gearboxBearingHolderForward:1
- Mate:1075: forwardBallastSealingWallFront:1 ↔ gearboxBearingHolderHexNutBacking:1
- Mate:1076: forwardBallastSealingWallFront:1 ↔ gearboxBearingHolderHexNutBacking:1
- Mate:1077: gearboxBearingHolderHexNutBacking:1
- Mate:1078: gearboxBearingHolderHexNutBacking:1 ↔ flatPlasticScrewSmall:68
- Flush:499: forwardBallastSealingWallFront:1 ↔ flatPlasticScrewSmall:68
- Mate:1079: gearboxBearingHolderHexNutBacking:1 ↔ flatPlasticScrewSmall:69
- Flush:500: forwardBallastSealingWallFront:1 ↔ flatPlasticScrewSmall:69
- Mate:1080: gearboxBearingHolderHexNutBacking:1 ↔ HexNutThread_M3:4
- Mate:1081: gearboxBearingHolderHexNutBacking:1 ↔ HexNutThread_M3:4
- Angle:74 (0 deg): gearboxBearingHolderHexNutBacking:1 ↔ HexNutThread_M3:4
- Mate:1082: gearboxBearingHolderHexNutBacking:1 ↔ HexNutThread_M3:5
- Mate:1083: gearboxBearingHolderHexNutBacking:1 ↔ HexNutThread_M3:5
- Angle:75 (0 deg): gearboxBearingHolderHexNutBacking:1 ↔ HexNutThread_M3:5
- Mate:1084: gearboxBearingHolderForward:1 ↔ Bolt_SocketHead_Hex_Thread_M3_8mm:1
- Mate:1085: gearboxBearingHolderForward:1 ↔ Bolt_SocketHead_Hex_Thread_M3_8mm:1
- Mate:1086: gearboxBearingHolderForward:1 ↔ Bolt_SocketHead_Hex_Thread_M3_8mm:2
- Mate:1087: gearboxBearingHolderForward:1 ↔ Bolt_SocketHead_Hex_Thread_M3_8mm:2
- Angle:76 (0 deg): Bolt_SocketHead_Hex_Thread_M3_8mm:2
- Angle:77 (0 deg): Bolt_SocketHead_Hex_Thread_M3_8mm:1
- Mate:1088: bearing_1_8inch:18 ↔ gearboxBearingHolderForward:1
- Mate:1089: forwardBallastSealingWallFront:1 ↔ bearing_1_8inch:18
- Mate:1090: forwardBallastSealingWallFront:1 ↔ idlerShaft2:2
- Mate:1091: bearing_1_8inch:17 ↔ gearboxBearingHolderForward:1
- Mate:1092: forwardBallastSealingWallFront:1 ↔ bearing_1_8inch:17
- Mate:1093: forwardBallastSealingWallFront:1 ↔ idlerShaft2:1
- Mate:1094 (0.127 mm): largeIdlerPinion:6 ↔ gearboxBearingHolderForward:1
- Mate:1095: bearing_1_8inch:16 ↔ gearboxBearingHolderForward:1
- Mate:1096: forwardBallastSealingWallFront:1 ↔ bearing_1_8inch:16
- Mate:1097: forwardBallastSealingWallFront:1 ↔ idlerShaft:1
- Mate:1099: forwardBallastSealingWallFront:1 ↔ pushSwitchRod:1
- Mate:1100: WeldNutThread_5_16_18:2 ↔ Bolt_ButtonHead_Hex_Thread_M3_10mm:1
- Mate:1101: WeldNutThread_5_16_18:2 ↔ Bolt_ButtonHead_Hex_Thread_M3_10mm:1
- Mate:1102: HexNutThread_M3:1 ↔ Bolt_ButtonHead_Hex_Thread_M3_10mm:3
- Mate:1103: GearMotorMountArm:1 ↔ aftServoSectionThreadedRodThread_5_40:1
- Mate:1104: GearMotorMount:1 ↔ GearMotorMountArm:1
- Flush:501: GearMotorMount:1 ↔ GearMotorMountArm:1
- Mate:1105 (0.254 mm): smallIdlerPinion:7 ↔ 3mm_.125inch_ShaftCoupler:1
- Mate:1106: NarrowHexNutThread_5_40:209 ↔ aftServoSectionThreadedRodThread_5_40:2
- Mate:1107: NarrowHexNutThread_5_40:210 ↔ aftServoSectionThreadedRodThread_5_40:2
- Angle:78 (0 deg): NarrowHexNutThread_5_40:209 ↔ NarrowHexNutThread_5_40:210
- Angle:79 (0 deg): ServoWithShaftAssembly:1 ↔ NarrowHexNutThread_5_40:210
- Mate:1108: NarrowHexNutThread_5_40:209 ↔ HallEffectSpoolSensorMount2:1